# Autodesk Inventor assembly: Drivetrain 2025-2026
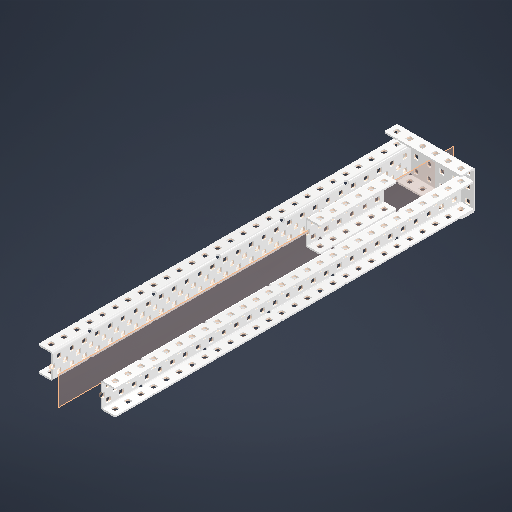
[picture p0: Inventor's stored thumbnail of the model, 512x512]
Saved by Autodesk Inventor 2026.2 (Build 302298000, 298)
## iProperties
Created: 2025-11-06
Part Number: Drivetrain 2025-2026
Document SubType Name: Assembly
Designer: thero
Author: thero
## Documents named in this file (5)
- C:\GitHub Repos\VEX-PushBack_2025-26\Push Back CAD\Drivetrain 2025-2026.iam
- C:\Users\thero\OneDrive\Desktop\VEX-CAD-Inventor-main\Structure\C Channel\Aluminum 1x2x1\Alu C 1x2x1x28.ipt
- C:\Users\thero\OneDrive\Desktop\VEX-CAD-Inventor-main\Structure\C Channel\Aluminum 1x2x1\Alu C 1x2x1x28_MIR.ipt
- C:\Users\thero\OneDrive\Desktop\VEX-CAD-Inventor-main\Structure\C Channel\Aluminum 1x3x1\Alu C 1x3x1x6.ipt
- C:\Users\thero\OneDrive\Desktop\VEX-CAD-Inventor-main\Structure\C Channel\Aluminum 1x2x1\Alu C 1x2x1x6.ipt
## Components (4 placed, 4 different names)
1. Alu C 1x2x1x28:1 — Flush:1, Insert:1, Insert:3, Insert:4
2. Alu C 1x2x1x28_MIR:1 — Mate:1, Insert:2
3. Alu C 1x3x1x6:1 — Insert:1, Insert:2
4. Alu C 1x2x1x6:1 — Insert:3, Insert:4
## Relationships (6: Insert 4, Flush 1, Mate 1)
- Flush:1 (-38.1 mm): Alu C 1x2x1x28:1
- Mate:1 (-38.1 mm): Alu C 1x2x1x28_MIR:1
- Insert:1: Alu C 1x2x1x28:1 ↔ Alu C 1x3x1x6:1
- Insert:2: Alu C 1x2x1x28_MIR:1 ↔ Alu C 1x3x1x6:1
- Insert:3 (12.7 mm): Alu C 1x2x1x28:1 ↔ Alu C 1x2x1x6:1
- Insert:4 (12.7 mm): Alu C 1x2x1x28:1 ↔ Alu C 1x2x1x6:1
